# Autodesk Inventor assembly: Assembly1
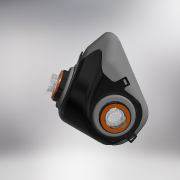
[picture p0: Inventor's stored thumbnail of the model, 180x180]
Saved by Autodesk Inventor 2021 (Build 250183000, 183)
## iProperties
Created: 2020-06-07
Part Number: Assembly1
Document SubType Name: Assembly
Designer: Derm
Author: Derm
## Documents named in this file (6)
- C:\Users\Derm\n95\v6\Assembly1.iam
- C:\Users\Derm\n95\v6\maskBody.ipt
- C:\Users\Derm\n95\v6\3dpBayonetteMountV2.ipt
- C:\Users\Derm\n95\v6\3dpBayonetteMountV1Fastener.ipt
- C:\Users\Derm\n95\v6\outerMountGasket.ipt
- C:\Users\Derm\n95\v6\overmoldStrapAnchor.ipt
## Components (8 placed, 5 different names)
1. maskBody:1 — Mate:1, Mate:2, Mate:3, Mate:4, Mate:12, Mate:15, Mate:18
2. 3dpBayonetteMountV2:1 — Mate:1, Mate:2, Mate:5, Mate:13
3. 3dpBayonetteMountV2:2 — Mate:3, Mate:4, Mate:6, Mate:9, Mate:12, Mate:14
4. 3dpBayonetteMountV1Fastener:1 — Mate:6, Mate:17, Mate:18
5. 3dpBayonetteMountV1Fastener:2 — Mate:5, Mate:7, Mate:15, Mate:16
6. outerMountGasket:1 — Mate:7, Mate:16
7. outerMountGasket:2 — Mate:9, Mate:17
8. overmoldStrapAnchor:1 — Mate:13, Mate:14
## Relationships (15: Mate 15)
- Mate:1: maskBody:1 ↔ 3dpBayonetteMountV2:1
- Mate:2: maskBody:1 ↔ 3dpBayonetteMountV2:1
- Mate:3: maskBody:1 ↔ 3dpBayonetteMountV2:2
- Mate:4: maskBody:1 ↔ 3dpBayonetteMountV2:2
- Mate:5: 3dpBayonetteMountV2:1 ↔ 3dpBayonetteMountV1Fastener:2
- Mate:6: 3dpBayonetteMountV2:2 ↔ 3dpBayonetteMountV1Fastener:1
- Mate:7: 3dpBayonetteMountV1Fastener:2 ↔ outerMountGasket:1
- Mate:9: 3dpBayonetteMountV2:2 ↔ outerMountGasket:2
- Mate:12: maskBody:1 ↔ 3dpBayonetteMountV2:2
- Mate:13: 3dpBayonetteMountV2:1 ↔ overmoldStrapAnchor:1
- Mate:14: 3dpBayonetteMountV2:2 ↔ overmoldStrapAnchor:1
- Mate:15: maskBody:1 ↔ 3dpBayonetteMountV1Fastener:2
- Mate:16: 3dpBayonetteMountV1Fastener:2 ↔ outerMountGasket:1
- Mate:17: 3dpBayonetteMountV1Fastener:1 ↔ outerMountGasket:2
- Mate:18: maskBody:1 ↔ 3dpBayonetteMountV1Fastener:1
